# Autodesk Inventor assembly: maskAssembly
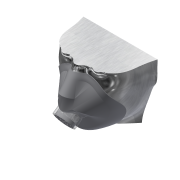
[picture p0: Inventor's stored thumbnail of the model, 180x180]
Saved by Autodesk Inventor 2018 (Build 220112000, 112)
## iProperties
Created: 2020-03-27
Part Number: maskAssembly
Document SubType Name: Assembly
Designer: Matt
Author: Matt
## Documents named in this file (5)
- C:\Users\Matt\n95\maskAssembly.iam
- C:\Users\Matt\n95\maskBodyV2.ipt
- C:\Users\Matt\n95\insideFlange.ipt
- C:\Users\Matt\n95\middleFlange.ipt
- C:\Users\Matt\n95\lid.ipt
## Components (4 placed, 4 different names)
1. maskBodyV2:1 — Mate:1
2. insideFlange:1 — Mate:1, Mate:2, Mate:3
3. middleFlange:1 — Mate:2, Mate:4
4. lid:1 — Mate:3, Mate:4
## Relationships (4: Mate 4)
- Mate:1: maskBodyV2:1 ↔ insideFlange:1
- Mate:2: insideFlange:1 ↔ middleFlange:1
- Mate:3: insideFlange:1 ↔ lid:1
- Mate:4: middleFlange:1 ↔ lid:1
